# Autodesk Inventor assembly: Сервопривод с кареткой
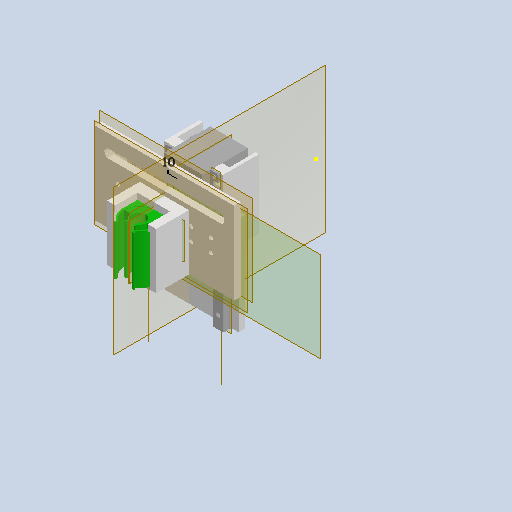
[picture p0: Inventor's stored thumbnail of the model, 512x512]
Saved by Autodesk Inventor 2024.2 (Build 282272000, 272)
## iProperties
Created: 2025-11-27
Part Number: Сервопривод с кареткой
Document SubType Name: Assembly
Designer: katya_notebook
Author: katya_notebook
## Documents named in this file (15)
- D:\alletz\construction\Сервопривод с кареткой.iam
- D:\alletz\construction\JX Servo PDI-HV2006MG\JX Servo PDI-HV2006MG.ipt
- D:\alletz\construction\MGN7C каретка\MGN7C каретка.ipt
- D:\alletz\construction\MHN7C рельса\MHN7C рельса.ipt
- D:\alletz\construction\крепление рельс.ipt
- D:\alletz\construction\крепление каретки.ipt
- D:\alletz\construction\подшипник мини.ipt
- D:\alletz\construction\деталь которая двигает.ipt
- D:\alletz\construction\деталь на которой рельсы.ipt
- D:\alletz\construction\25T Servo Horn Steering Arm M3 версия 3.ipt
- D:\alletz\construction\держатель сервомоторчика.ipt
- D:\alletz\construction\крепление маркера 8мм.ipt
- D:\alletz\construction\держатель магнитов на основе.ipt
- D:\alletz\construction\крепление маркера 18мм.ipt
- D:\alletz\construction\проставк.ipt
## Components (17 placed, 14 different names)
1. JX Servo PDI-HV2006MG:1 — Совмещение:5, Совмещение:9, Совмещение:10, С поворотом:1, Совмещение:11, Заподлицо:5
2. MGN7C каретка:1 — Жесткий:2, Совмещение:8, Совмещение:14, С поворотом:2
3. MHN7C рельса:1 — Совмещение:2, Заподлицо:1, Совмещение:3, Совмещение:4, Жесткий:2, Совмещение:6, Совмещение:7, Заподлицо:3
4. крепление рельс:1
5. крепление каретки:1
6. подшипник мини:1 — Совмещение:12
7. MHN7C рельса:2 — Заподлицо:1, Совмещение:3, Совмещение:6, Совмещение:7, Жесткий:3
8. MGN7C каретка:2 — Жесткий:3, Совмещение:8, Заподлицо:4, Совмещение:11, Совмещение:13
9. деталь которая двигает:1 — Заподлицо:3
10. деталь на которой рельсы:1 — Заподлицо:4, Совмещение:9, Заподлицо:6, Заподлицо:8, Заподлицо:9, Совмещение:15
11. 25T Servo Horn Steering Arm M3 версия 3:1 — Совмещение:10, С поворотом:1, Совмещение:12
12. держатель сервомоторчика:1 — Заподлицо:5
13. крепление маркера 8мм:1 — Заподлицо:6, Совмещение:17, Совмещение:18
14. держатель магнитов на основе:1 — Заподлицо:8, Заподлицо:9, Совмещение:15, Совмещение:16, Совмещение:18, Совмещение:19
15. крепление маркера 18мм:1 — Совмещение:16, Совмещение:17, Совмещение:19
16. проставк:1 — Совмещение:13
17. проставк:2 — Совмещение:14, С поворотом:2
## Relationships (29: Mate 18, Flush 7, WeldJoint 2, RevoluteJoint 2)
- Совмещение:2 [Mate]: MHN7C рельса:1
- Заподлицо:1 [Flush]: MHN7C рельса:1 ↔ MHN7C рельса:2
- Совмещение:3 [Mate] (38 mm): MHN7C рельса:1 ↔ MHN7C рельса:2
- Совмещение:4 [Mate] (22.3 mm): MHN7C рельса:1
- Совмещение:5 [Mate]: JX Servo PDI-HV2006MG:1
- Жесткий:2 [WeldJoint]: MGN7C каретка:1 ↔ MHN7C рельса:1
- Совмещение:6 [Mate]: MHN7C рельса:1 ↔ MHN7C рельса:2
- Совмещение:7 [Mate]: MHN7C рельса:1 ↔ MHN7C рельса:2
- Жесткий:3 [WeldJoint]: MHN7C рельса:2 ↔ MGN7C каретка:2
- Совмещение:8 [Mate]: MGN7C каретка:1 ↔ MGN7C каретка:2
- Заподлицо:3 [Flush]: MHN7C рельса:1 ↔ деталь которая двигает:1
- Заподлицо:4 [Flush]: MGN7C каретка:2 ↔ деталь на которой рельсы:1
- Совмещение:9 [Mate] (7.5 mm): JX Servo PDI-HV2006MG:1 ↔ деталь на которой рельсы:1
- Совмещение:10 [Mate]: JX Servo PDI-HV2006MG:1 ↔ 25T Servo Horn Steering Arm M3 версия 3:1
- С поворотом:1 [RevoluteJoint]: JX Servo PDI-HV2006MG:1 ↔ 25T Servo Horn Steering Arm M3 версия 3:1
- Совмещение:11 [Mate]: JX Servo PDI-HV2006MG:1 ↔ MGN7C каретка:2
- Совмещение:12 [Mate]: подшипник мини:1 ↔ 25T Servo Horn Steering Arm M3 версия 3:1
- Заподлицо:5 [Flush]: JX Servo PDI-HV2006MG:1 ↔ держатель сервомоторчика:1
- Заподлицо:6 [Flush]: деталь на которой рельсы:1 ↔ крепление маркера 8мм:1
- Заподлицо:8 [Flush]: деталь на которой рельсы:1 ↔ держатель магнитов на основе:1
- Заподлицо:9 [Flush] (-27.55 mm): деталь на которой рельсы:1 ↔ держатель магнитов на основе:1
- Совмещение:13 [Mate]: MGN7C каретка:2 ↔ проставк:1
- Совмещение:14 [Mate]: MGN7C каретка:1 ↔ проставк:2
- С поворотом:2 [RevoluteJoint]: MGN7C каретка:1 ↔ проставк:2
- Совмещение:15 [Mate]: деталь на которой рельсы:1 ↔ держатель магнитов на основе:1
- Совмещение:16 [Mate]: держатель магнитов на основе:1 ↔ крепление маркера 18мм:1
- Совмещение:17 [Mate]: крепление маркера 8мм:1 ↔ крепление маркера 18мм:1
- Совмещение:18 [Mate] (0.2 mm): крепление маркера 8мм:1 ↔ держатель магнитов на основе:1
- Совмещение:19 [Mate] (0.2 mm): держатель магнитов на основе:1 ↔ крепление маркера 18мм:1
